# Autodesk Inventor assembly: CyberOrto
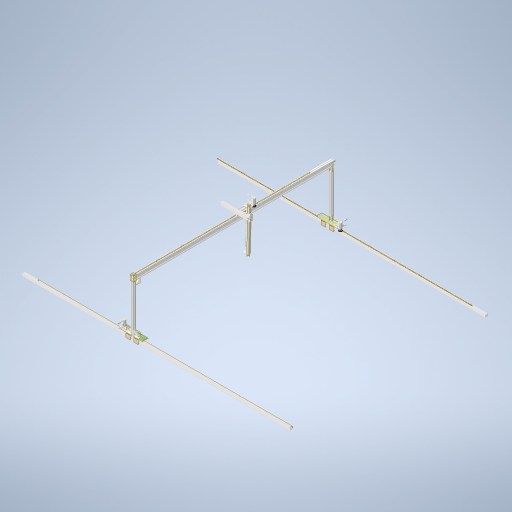
[picture p0: Inventor's stored thumbnail of the model, 512x512]
Saved by Autodesk Inventor 2023 (Build 270158000, 158)
## iProperties
RuleStatus: InUse
Created: 2021-12-29
Part Number: CyberOrto
Document SubType Name: Assembly
Designer: matte
Author: matte
## Documents named in this file (23)
- C:\Users\matte\Documents\GitHub\MDM-CyberOrto-CAD\CyberOrto.iam
- C:\Users\matte\Documents\GitHub\MDM-CyberOrto-CAD\Pezzi singoli\Supporto SX.ipt
- C:\Users\matte\Documents\GitHub\MDM-CyberOrto-CAD\Parker components\03-Brackets_Gussets_Plates\09-Machined Gussets\20-102.ipt
- C:\Users\matte\Documents\GitHub\MDM-CyberOrto-CAD\Parker components\02-Fasteners\10-Standard T-Nuts\20-050.ipt
- C:\Users\matte\Documents\GitHub\MDM-CyberOrto-CAD\Parker components\02-Fasteners\16-Screws\01-Metric Screws\01-Button Head\24-118-8.ipt
- C:\Users\matte\Documents\GitHub\MDM-CyberOrto-CAD\Guida a terra.iam
- C:\Users\matte\Documents\GitHub\MDM-CyberOrto-CAD\Parker components\05-Handles_Hinges\13-Pivot Joints\23-010.iam
- C:\Users\matte\Documents\GitHub\MDM-CyberOrto-CAD\Parker components\02-Fasteners\10-Standard T-Nuts\20-058.ipt
- C:\Users\matte\Documents\GitHub\MDM-CyberOrto-CAD\Parker components\02-Fasteners\16-Screws\01-Metric Screws\01-Button Head\24-116-8.ipt
- C:\Users\matte\Documents\GitHub\MDM-CyberOrto-CAD\Pezzi singoli\Supporto DX.ipt
- C:\Users\matte\Documents\GitHub\MDM-CyberOrto-CAD\Parker components\02-Fasteners\16-Screws\01-Metric Screws\01-Button Head\24-120-8.ipt
- C:\Users\matte\Documents\GitHub\MDM-CyberOrto-CAD\Pezzi singoli\Supporto lineare\Carrello semplice.iam
- C:\Users\matte\Documents\GitHub\MDM-CyberOrto-CAD\Rack_Pinion\pinion_scaled1.ipt
- C:\Users\matte\Documents\GitHub\MDM-CyberOrto-CAD\Trave a terra\Trave a terra.iam
- C:\Users\matte\Documents\GitHub\MDM-CyberOrto-CAD\Torretta.iam
- C:\Users\matte\Documents\GitHub\MDM-CyberOrto-CAD\Pezzi singoli\13-106_f.ipt
- C:\Users\matte\Documents\GitHub\MDM-CyberOrto-CAD\Pezzi singoli\13-513.ipt
- C:\Users\matte\Documents\GitHub\MDM-CyberOrto-CAD\Rack_Pinion\Rack_series.iam
- C:\Users\matte\Documents\GitHub\MDM-CyberOrto-CAD\Rack_Pinion\Motor_assembly.iam
- C:\Users\matte\Documents\GitHub\MDM-CyberOrto-CAD\Rack_Pinion\Rack_series_upper.iam
- C:\Users\matte\Documents\GitHub\MDM-CyberOrto-CAD\Rack_Pinion\Rack_truncated.iam
- C:\Users\matte\Documents\GitHub\MDM-CyberOrto-CAD\Parker components\02-Fasteners\16-Screws\01-Metric Screws\03-Socket Head\24-320-4.ipt
- C:\Users\matte\Documents\GitHub\MDM-CyberOrto-CAD\Pezzi singoli\10-080.ipt
## Components (37 placed, 22 different names)
1. Supporto SX:1 — Coincidente:6, Allineato:3, Coincidente:7, Coincidente:15, Coincidente:16, Coincidente:23, Coincidente:28, Coincidente:29, Coincidente:30, Allineato:159, Coincidente:280, Allineato:160, Allineato:164
2. Supporto DX:1 — Coincidente:45, Allineato:7, Allineato:8, Coincidente:48, Allineato:9, Allineato:10
3. Torretta:1 [sub-assembly] — Coincidente:258, Allineato:145, Coincidente:284
4. pinion_scaled1:3 — Coincidente:258
5. 13-106_f:1 — Coincidente:264, Allineato:145, Allineato:162, Allineato:164, Coincidente:281, Allineato:166
6. 13-106_f:2 — Coincidente:263, Allineato:161, Coincidente:282, Allineato:166, Allineato:167
7. 13-513:1 — Coincidente:264, Allineato:162, Allineato:163
8. 13-513:2 — Coincidente:263, Allineato:161, Allineato:163
9. Rack_series:1 [sub-assembly] — Coincidente:272, Angolo:9, Allineato:150, Allineato:151
10. Rack_series:2 [sub-assembly] — Coincidente:273, Allineato:152, Allineato:153
11. Motor_assembly:1 [sub-assembly] — Coincidente:274, Allineato:154, Allineato:155
12. Rack_series_upper:1 [sub-assembly] — Coincidente:276, Allineato:158, Coincidente:278, Coincidente:279, Coincidente:283
13. Rack_truncated:1 [sub-assembly] — Coincidente:276, Allineato:158
14. 24-320-4:1 — Coincidente:278, Coincidente:279
15. 10-080:1 — Allineato:159, Coincidente:280, Allineato:160, Coincidente:281, Coincidente:282, Allineato:167, Coincidente:283, Coincidente:284
16. 24-118-8:3 — Coincidente:19, Coincidente:20
17. 24-118-8:4 — Coincidente:21, Coincidente:22
18. 20-050:2 — Coincidente:11, Coincidente:12
19. 24-118-8:1 — Coincidente:13, Coincidente:14
20. 24-118-8:2 — Coincidente:17, Coincidente:18
21. 20-102:1 — Coincidente:6, Allineato:3, Coincidente:8, Coincidente:9, Coincidente:11, Coincidente:12, Coincidente:13, Coincidente:14, Coincidente:17, Coincidente:18, Coincidente:19, Coincidente:20, Coincidente:21, Coincidente:22
22. 20-050:1 — Coincidente:7, Coincidente:8, Coincidente:9
23. 24-118-8:5 — Coincidente:31, Coincidente:32, Coincidente:33
24. 24-118-8:6 — Coincidente:34, Coincidente:35
25. 24-118-8:7 — Coincidente:38, Coincidente:39
26. 24-118-8:8 — Coincidente:36, Coincidente:37
27. Guida a terra:1 [sub-assembly] — Coincidente:15, Coincidente:16, Coincidente:23, Coincidente:32, Coincidente:33, Coincidente:34, Coincidente:35, Coincidente:36, Coincidente:37, Coincidente:38, Coincidente:39, Coincidente:210, Allineato:115, Coincidente:274, Allineato:154, Allineato:155
28. 20-050:3 — Coincidente:27, Allineato:4, Coincidente:28, Coincidente:30, Coincidente:31
29. 20-050:4 — Coincidente:27, Allineato:4, Coincidente:29
30. 23-010:1 [sub-assembly] — Coincidente:43, Coincidente:44, Coincidente:45, Allineato:7, Allineato:8, Coincidente:46, Coincidente:47
31. 20-058:1 — Coincidente:42
32. 24-116-8:1 — Coincidente:42, Coincidente:43, Coincidente:44
33. 24-120-8:1 — Coincidente:46, Coincidente:47
34. 24-120-8:2 — Coincidente:51, Coincidente:52
35. Carrello semplice:1 [sub-assembly] — Coincidente:48, Allineato:9, Allineato:10, Coincidente:51, Coincidente:52, Angolo:2, Angolo:3, Angolo:4, Allineato:59, Coincidente:130
36. Trave a terra:1 [sub-assembly] — Angolo:2, Angolo:3, Angolo:4, Allineato:59, Coincidente:130, Allineato:149, Coincidente:272, Angolo:9, Allineato:150, Allineato:151
37. Trave a terra:2 [sub-assembly] — Coincidente:210, Allineato:115, Allineato:149, Coincidente:273, Allineato:152, Allineato:153
## Relationships (84: Mate 55, Flush 25, Angle 4)
- Coincidente:6 [Mate]: Supporto SX:1 ↔ 20-102:1
- Allineato:3 [Flush]: Supporto SX:1 ↔ 20-102:1
- Coincidente:7 [Mate]: Supporto SX:1 ↔ 20-050:1
- Coincidente:8 [Mate]: 20-102:1 ↔ 20-050:1
- Coincidente:9 [Mate]: 20-102:1 ↔ 20-050:1
- Coincidente:11 [Mate]: 20-050:2 ↔ 20-102:1
- Coincidente:12 [Mate]: 20-050:2 ↔ 20-102:1
- Coincidente:13 [Mate]: 24-118-8:1 ↔ 20-102:1
- Coincidente:14 [Mate]: 24-118-8:1 ↔ 20-102:1
- Coincidente:15 [Mate]: Supporto SX:1 ↔ Guida a terra:1
- Coincidente:16 [Mate]: Supporto SX:1 ↔ Guida a terra:1
- Coincidente:17 [Mate]: 24-118-8:2 ↔ 20-102:1
- Coincidente:18 [Mate]: 24-118-8:2 ↔ 20-102:1
- Coincidente:19 [Mate]: 24-118-8:3 ↔ 20-102:1
- Coincidente:20 [Mate]: 24-118-8:3 ↔ 20-102:1
- Coincidente:21 [Mate]: 24-118-8:4 ↔ 20-102:1
- Coincidente:22 [Mate]: 24-118-8:4 ↔ 20-102:1
- Coincidente:23 [Mate]: Supporto SX:1 ↔ Guida a terra:1
- Coincidente:27 [Mate]: 20-050:3 ↔ 20-050:4
- Allineato:4 [Flush]: 20-050:3 ↔ 20-050:4
- Coincidente:28 [Mate]: Supporto SX:1 ↔ 20-050:3
- Coincidente:29 [Mate]: Supporto SX:1 ↔ 20-050:4
- Coincidente:30 [Mate]: Supporto SX:1 ↔ 20-050:3
- Coincidente:31 [Mate]: 24-118-8:5 ↔ 20-050:3
- Coincidente:32 [Mate]: 24-118-8:5 ↔ Guida a terra:1
- Coincidente:33 [Mate]: 24-118-8:5 ↔ Guida a terra:1
- Coincidente:34 [Mate]: 24-118-8:6 ↔ Guida a terra:1
- Coincidente:35 [Mate]: 24-118-8:6 ↔ Guida a terra:1
- Coincidente:36 [Mate]: 24-118-8:8 ↔ Guida a terra:1
- Coincidente:37 [Mate]: 24-118-8:8 ↔ Guida a terra:1
- Coincidente:38 [Mate]: 24-118-8:7 ↔ Guida a terra:1
- Coincidente:39 [Mate]: 24-118-8:7 ↔ Guida a terra:1
- Coincidente:42 [Mate]: 20-058:1 ↔ 24-116-8:1
- Coincidente:43 [Mate]: 23-010:1 ↔ 24-116-8:1
- Coincidente:44 [Mate]: 23-010:1 ↔ 24-116-8:1
- Coincidente:45 [Mate]: Supporto DX:1 ↔ 23-010:1
- Allineato:7 [Flush]: Supporto DX:1 ↔ 23-010:1
- Allineato:8 [Flush]: Supporto DX:1 ↔ 23-010:1
- Coincidente:46 [Mate]: 23-010:1 ↔ 24-120-8:1
- Coincidente:47 [Mate]: 23-010:1 ↔ 24-120-8:1
- Coincidente:48 [Mate]: Supporto DX:1 ↔ Carrello semplice:1
- Allineato:9 [Flush]: Supporto DX:1 ↔ Carrello semplice:1
- Allineato:10 [Flush]: Supporto DX:1 ↔ Carrello semplice:1
- Coincidente:51 [Mate]: 24-120-8:2 ↔ Carrello semplice:1
- Coincidente:52 [Mate]: 24-120-8:2 ↔ Carrello semplice:1
- Angolo:2 [Angle] (0 deg): Carrello semplice:1 ↔ Trave a terra:1
- Angolo:3 [Angle] (0 deg): Carrello semplice:1 ↔ Trave a terra:1
- Angolo:4 [Angle] (0 deg): Carrello semplice:1 ↔ Trave a terra:1
- Allineato:59 [Flush] (19 mm): Carrello semplice:1 ↔ Trave a terra:1
- Coincidente:130 [Mate] (20 mm): Carrello semplice:1 ↔ Trave a terra:1
- Coincidente:210 [Mate] (20 mm): Guida a terra:1 ↔ Trave a terra:2
- Allineato:115 [Flush] (19 mm): Guida a terra:1 ↔ Trave a terra:2
- Coincidente:258 [Mate]: Torretta:1 ↔ pinion_scaled1:3
- Coincidente:263 [Mate]: 13-106_f:2 ↔ 13-513:2
- Coincidente:264 [Mate]: 13-106_f:1 ↔ 13-513:1
- Allineato:145 [Flush] (19 mm): Torretta:1 ↔ 13-106_f:1
- Allineato:149 [Flush]: Trave a terra:1 ↔ Trave a terra:2
- Coincidente:272 [Mate]: Rack_series:1 ↔ Trave a terra:1
- Angolo:9 [Angle] (0 deg): Rack_series:1 ↔ Trave a terra:1
- Allineato:150 [Flush]: Rack_series:1 ↔ Trave a terra:1
- Allineato:151 [Flush] (12.5 mm): Rack_series:1 ↔ Trave a terra:1
- Coincidente:273 [Mate]: Rack_series:2 ↔ Trave a terra:2
- Allineato:152 [Flush]: Rack_series:2 ↔ Trave a terra:2
- Allineato:153 [Flush] (12.5 mm): Rack_series:2 ↔ Trave a terra:2
- Coincidente:274 [Mate]: Motor_assembly:1 ↔ Guida a terra:1
- Allineato:154 [Flush]: Motor_assembly:1 ↔ Guida a terra:1
- Allineato:155 [Flush] (10 mm): Motor_assembly:1 ↔ Guida a terra:1
- Coincidente:276 [Mate]: Rack_series_upper:1 ↔ Rack_truncated:1
- Allineato:158 [Flush]: Rack_series_upper:1 ↔ Rack_truncated:1
- Coincidente:278 [Mate]: Rack_series_upper:1 ↔ 24-320-4:1
- Coincidente:279 [Mate]: Rack_series_upper:1 ↔ 24-320-4:1
- Allineato:159 [Flush]: Supporto SX:1 ↔ 10-080:1
- Coincidente:280 [Mate]: Supporto SX:1 ↔ 10-080:1
- Allineato:160 [Flush]: Supporto SX:1 ↔ 10-080:1
- Allineato:161 [Flush]: 13-106_f:2 ↔ 13-513:2
- Allineato:162 [Flush]: 13-106_f:1 ↔ 13-513:1
- Allineato:163 [Flush]: 13-513:1 ↔ 13-513:2
- Allineato:164 [Flush]: Supporto SX:1 ↔ 13-106_f:1
- Coincidente:281 [Mate]: 13-106_f:1 ↔ 10-080:1
- Coincidente:282 [Mate]: 13-106_f:2 ↔ 10-080:1
- Allineato:166 [Flush]: 13-106_f:1 ↔ 13-106_f:2
- Allineato:167 [Flush] (13.5 mm): 13-106_f:2 ↔ 10-080:1
- Coincidente:283 [Mate]: Rack_series_upper:1 ↔ 10-080:1
- Coincidente:284 [Mate] (20 mm): Torretta:1 ↔ 10-080:1
